# Autodesk Inventor assembly: Assembly146-01
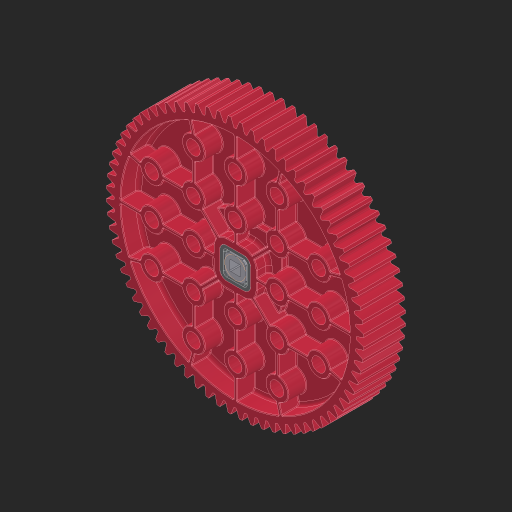
[picture p0: Inventor's stored thumbnail of the model, 512x512]
Saved by Autodesk Inventor 2023 (Build 270158000, 158)
## iProperties
Created: 2022-08-02
Part Number: Assembly146-01
Document SubType Name: Assembly
Designer: ylu12
Author: ylu12
## Documents named in this file (4)
- C:\Users\ylu12\Documents\GitHub\VEX-CAD-Inventor\Motion\Gears\HS Gear\HS 72T Gear, Square.iam
- C:\Users\ylu12\Documents\GitHub\VEX-CAD-Inventor\Motion\HS Shaft Adapter Square.ipt
- C:\Users\ylu12\Documents\GitHub\VEX-CAD-Inventor\Motion\Gears\Reference Files\HS 72T Gear, No Insert.ipt
- C:\Users\ylu12\Documents\GitHub\VEX-CAD-Inventor\Motion\Gears\HS Gear.iam
## Components (2 placed, 2 different names)
1. Square — Mate:3, Mate:4, Flush:2
2. 72T — Flush:8, Mate:15, Mate:16
## Relationships (6: Mate 4, Flush 2)
- Mate:3: Square
- Mate:4: Square
- Flush:2 (6.35 mm): Square
- Flush:8: 72T
- Mate:15: 72T
- Mate:16: 72T
